# Autodesk Inventor assembly: AS_GENERAL
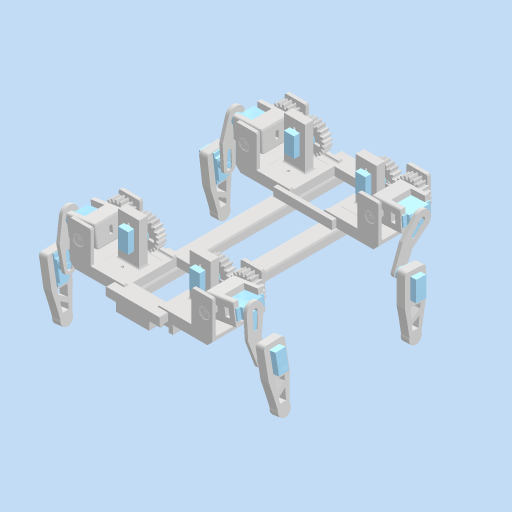
[picture p0: Inventor's stored thumbnail of the model, 512x512]
Saved by Autodesk Inventor 2024 (Build 280153000, 153)
## iProperties
Created: 2024-09-28
Part Number: AS_GENERAL
Document SubType Name: Assembly
Designer: MxMon
Author: MxMon
## Documents named in this file (22)
- C:\Users\MxMon\Documents\Inventor\CHEWIETRON\AS_GENERAL.iam
- C:\Users\MxMon\Documents\Inventor\CHEWIETRON\BASEPRINCIPAL_PATA_IZQ.ipt
- C:\Users\MxMon\Documents\Inventor\CHEWIETRON\bearing_604zz\bearing_604zz.ipt
- C:\Users\MxMon\Documents\Inventor\CHEWIETRON\BASEMOTOR_HOMBRO.ipt
- C:\Users\MxMon\Documents\Inventor\CHEWIETRON\Servo mockup\Servo mockup.ipt
- C:\Users\MxMon\Documents\Inventor\CHEWIETRON\Servo Motor hélice\Servo Motor hélice.ipt
- C:\Users\MxMon\Documents\Inventor\CHEWIETRON\PATA_SUP_IZQ.ipt
- C:\Users\MxMon\Documents\Inventor\CHEWIETRON\PARA_INF.ipt
- C:\Users\MxMon\Documents\Inventor\CHEWIETRON\BASEMOTOR_ENGRANE.ipt
- C:\Users\MxMon\Documents\Inventor\CHEWIETRON\CONECTOR_ENGRANE_HOMBRO.ipt
- C:\Users\MxMon\Documents\Inventor\CHEWIETRON\ENGRANE_HOMBRO.ipt
- C:\Users\MxMon\Documents\Inventor\CHEWIETRON\HELICE_CRUZ.ipt
- C:\Users\MxMon\Documents\Inventor\CHEWIETRON\ENGRANE_HELICE.ipt
- C:\Users\MxMon\Documents\Inventor\CHEWIETRON\EJE_TORNILLO.ipt
- C:\Users\MxMon\Documents\Inventor\CHEWIETRON\TUERCA.ipt
- C:\Users\MxMon\Documents\Inventor\CHEWIETRON\ESPACIADOR.ipt
- C:\Users\MxMon\Documents\Inventor\CHEWIETRON\BASE_DE_PRUEBA.ipt
- C:\Users\MxMon\Documents\Inventor\CHEWIETRON\BASEPRINCIPAL_PATA_DER.ipt
- C:\Users\MxMon\Documents\Inventor\CHEWIETRON\PATA_SUP_DER.ipt
- C:\Users\MxMon\Documents\Inventor\CHEWIETRON\UNION_CHEWIE.ipt
- C:\Users\MxMon\Documents\Inventor\CHEWIETRON\UNION_INTERNA.ipt
- C:\Users\MxMon\Documents\Inventor\CHEWIETRON\TAG.ipt
## Components (83 placed, 21 different names)
1. BASEPRINCIPAL_PATA_IZQ:1 — Mate:1, Mate:2, Mate:3, Mate:4, Mate:23, Mate:25, Mate:46, Mate:98, Mate:129, Mate:149, Flush:2, Mate:150, Mate:201, Mate:202, Mate:210, Mate:211
2. bearing_604zz:1 — Mate:1, Mate:2, Mate:5, Mate:39, Mate:40
3. bearing_604zz:2 — Mate:3, Mate:4, Mate:44
4. BASEMOTOR_HOMBRO:1 — Mate:5, Mate:6, Mate:7, Mate:8, Mate:26, Mate:27, Mate:28, Mate:42
5. Servo mockup:1 — Mate:6, Mate:7, Mate:8, Mate:9, Mate:10
6. Servo Motor hélice:1 — Mate:9, Mate:10, Mate:11, Mate:12, Mate:13
7. PATA_SUP_IZQ:1 — Mate:11, Mate:12, Mate:13, Mate:47, Mate:48, Mate:49, Mate:50
8. Servo mockup:2 — Mate:20, Mate:21, Mate:22
9. Servo Motor hélice:2 — Mate:47, Mate:48, Mate:49, Mate:50
10. PARA_INF:1 — Mate:20, Mate:21, Mate:22
11. BASEMOTOR_ENGRANE:1 — Mate:23, Mate:25, Mate:36, Mate:37, Mate:38, Mate:46
12. CONECTOR_ENGRANE_HOMBRO:1 — Mate:26, Mate:27, Mate:28, Mate:29, Mate:30, Mate:31
13. ENGRANE_HOMBRO:1 — Mate:29, Mate:30, Mate:31
14. Servo mockup:3 — Mate:32, Mate:33, Mate:36, Mate:37, Mate:38
15. HELICE_CRUZ:1 — Mate:32, Mate:33, Mate:34, Mate:35
16. ENGRANE_HELICE:1 — Mate:34, Mate:35
17. EJE_TORNILLO:1 — Mate:39, Mate:40, Mate:41, Mate:43
18. TUERCA:1 — Mate:41, Mate:42, Mate:45
19. ESPACIADOR:1 — Mate:43, Mate:44, Mate:45
20. BASEPRINCIPAL_PATA_IZQ:2 — Mate:97, Mate:99, Flush:1, Mate:130, Mate:131, Mate:205, Mate:206, Mate:212, Mate:213, Mate:214, Mate:216
21. bearing_604zz:3
22. bearing_604zz:4
23. BASEMOTOR_HOMBRO:2
24. Servo mockup:4
25. Servo Motor hélice:3
26. PATA_SUP_IZQ:2
27. Servo mockup:5
28. Servo Motor hélice:4
29. PARA_INF:2
30. BASEMOTOR_ENGRANE:2
31. CONECTOR_ENGRANE_HOMBRO:2
32. ENGRANE_HOMBRO:2
33. Servo mockup:6
34. HELICE_CRUZ:2
35. ENGRANE_HELICE:2
36. EJE_TORNILLO:2
37. TUERCA:2
38. ESPACIADOR:2
39. BASE_DE_PRUEBA:1 — Mate:97, Mate:98, Mate:99, Mate:129
40. BASEPRINCIPAL_PATA_DER:1 — Flush:1, Mate:101, Mate:102, Mate:103, Mate:111, Mate:112, Mate:113, Mate:114, Mate:130, Mate:131, Mate:207, Mate:215
41. BASEMOTOR_ENGRANE:3 — Mate:101, Mate:102, Mate:103, Mate:104, Mate:105, Mate:106
42. Servo mockup:7 — Mate:104, Mate:105, Mate:106, Mate:107, Mate:108
43. HELICE_CRUZ:3 — Mate:107, Mate:108, Mate:109, Mate:110
44. ENGRANE_HELICE:3 — Mate:109, Mate:110
45. bearing_604zz:5 — Mate:111, Mate:112, Mate:116
46. bearing_604zz:6 — Mate:113, Mate:114, Mate:115, Mate:132
47. EJE_TORNILLO:3 — Mate:115, Mate:116, Mate:124, Mate:125, Mate:127
48. BASEMOTOR_HOMBRO:3 — Mate:118, Mate:119, Mate:120, Mate:124, Mate:126, Mate:133, Mate:134, Mate:137
49. CONECTOR_ENGRANE_HOMBRO:3 — Mate:118, Mate:119, Mate:120, Mate:121, Mate:122, Mate:123
50. ENGRANE_HOMBRO:3 — Mate:121, Mate:122, Mate:123
51. TUERCA:3 — Mate:125, Mate:126, Mate:128
52. ESPACIADOR:3 — Mate:127, Mate:128, Mate:132
53. Servo mockup:8 — Mate:133, Mate:134, Mate:135, Mate:136, Mate:137
54. Servo Motor hélice:5 — Mate:135, Mate:136, Mate:138, Mate:139, Mate:140
55. PATA_SUP_DER:1 — Mate:138, Mate:139, Mate:140, Mate:143, Mate:144, Mate:145
56. Servo mockup:9 — Mate:146, Mate:147, Mate:148
57. Servo Motor hélice:6 — Mate:143, Mate:144, Mate:145
58. PARA_INF:3 — Mate:146, Mate:147, Mate:148
59. BASEPRINCIPAL_PATA_DER:2 — Mate:149, Flush:2, Mate:150, Mate:151, Mate:152, Mate:153, Mate:161, Mate:164, Mate:165, Mate:197, Mate:198, Mate:199, Mate:203, Mate:204, Mate:208, Mate:209
60. BASEMOTOR_ENGRANE:4 — Mate:151, Mate:152, Mate:153, Mate:154, Mate:155, Mate:156
61. Servo mockup:10 — Mate:154, Mate:155, Mate:156, Mate:157, Mate:158
62. HELICE_CRUZ:4 — Mate:157, Mate:158, Mate:159, Mate:160
63. ENGRANE_HELICE:4 — Mate:159, Mate:160
64. EJE_TORNILLO:4 — Mate:161, Mate:162, Mate:163, Mate:166, Mate:167, Mate:174, Mate:176
65. bearing_604zz:7 — Mate:163, Mate:165, Mate:166
66. bearing_604zz:8 — Mate:162, Mate:164, Mate:178
67. BASEMOTOR_HOMBRO:4 — Mate:167, Mate:168, Mate:169, Mate:170, Mate:175, Mate:183, Mate:184, Mate:185
68. CONECTOR_ENGRANE_HOMBRO:4 — Mate:168, Mate:169, Mate:170, Mate:171, Mate:172, Mate:173
69. ENGRANE_HOMBRO:4 — Mate:171, Mate:172, Mate:173
70. TUERCA:4 — Mate:174, Mate:175, Mate:177
71. ESPACIADOR:4 — Mate:176, Mate:177, Mate:178
72. Servo mockup:11 — Mate:181, Mate:182, Mate:183, Mate:184, Mate:185
73. PATA_SUP_DER:2 — Mate:186, Mate:187, Mate:188, Mate:191, Mate:192, Mate:193
74. Servo Motor hélice:7 — Mate:181, Mate:182, Mate:186, Mate:187, Mate:188
75. Servo mockup:12 — Mate:194, Mate:195, Mate:196
76. Servo Motor hélice:8 — Mate:191, Mate:192, Mate:193
77. PARA_INF:4 — Mate:194, Mate:195, Mate:196
78. BASE_DE_PRUEBA:2 — Mate:197, Mate:198, Mate:199
79. UNION_CHEWIE:1 — Mate:201, Mate:202, Mate:203, Mate:204, Mate:217, Mate:218, Mate:219
80. UNION_INTERNA:1 — Mate:205, Mate:206, Mate:207, Mate:212
81. UNION_INTERNA:2 — Mate:208, Mate:209, Mate:210, Mate:211
82. UNION_CHEWIE:2 — Mate:213, Mate:214, Mate:215, Mate:216
83. TAG:1 — Mate:217, Mate:218, Mate:219
## Relationships (210: Mate 208, Flush 2)
- Mate:1: BASEPRINCIPAL_PATA_IZQ:1 ↔ bearing_604zz:1
- Mate:2: BASEPRINCIPAL_PATA_IZQ:1 ↔ bearing_604zz:1
- Mate:3: BASEPRINCIPAL_PATA_IZQ:1 ↔ bearing_604zz:2
- Mate:4: BASEPRINCIPAL_PATA_IZQ:1 ↔ bearing_604zz:2
- Mate:5: bearing_604zz:1 ↔ BASEMOTOR_HOMBRO:1
- Mate:6: BASEMOTOR_HOMBRO:1 ↔ Servo mockup:1
- Mate:7: BASEMOTOR_HOMBRO:1 ↔ Servo mockup:1
- Mate:8: BASEMOTOR_HOMBRO:1 ↔ Servo mockup:1
- Mate:9: Servo mockup:1 ↔ Servo Motor hélice:1
- Mate:10: Servo mockup:1 ↔ Servo Motor hélice:1
- Mate:11: Servo Motor hélice:1 ↔ PATA_SUP_IZQ:1
- Mate:12: Servo Motor hélice:1 ↔ PATA_SUP_IZQ:1
- Mate:13: Servo Motor hélice:1 ↔ PATA_SUP_IZQ:1
- [Mate]: Servo mockup:2 ↔ Servo Motor hélice:2
- [Mate]: Servo mockup:2 ↔ Servo Motor hélice:2
- Mate:20: Servo mockup:2 ↔ PARA_INF:1
- Mate:21: Servo mockup:2 ↔ PARA_INF:1
- Mate:22: Servo mockup:2 ↔ PARA_INF:1
- Mate:23: BASEPRINCIPAL_PATA_IZQ:1 ↔ BASEMOTOR_ENGRANE:1
- Mate:25: BASEPRINCIPAL_PATA_IZQ:1 ↔ BASEMOTOR_ENGRANE:1
- Mate:26: BASEMOTOR_HOMBRO:1 ↔ CONECTOR_ENGRANE_HOMBRO:1
- Mate:27: BASEMOTOR_HOMBRO:1 ↔ CONECTOR_ENGRANE_HOMBRO:1
- Mate:28: BASEMOTOR_HOMBRO:1 ↔ CONECTOR_ENGRANE_HOMBRO:1
- Mate:29: CONECTOR_ENGRANE_HOMBRO:1 ↔ ENGRANE_HOMBRO:1
- Mate:30: CONECTOR_ENGRANE_HOMBRO:1 ↔ ENGRANE_HOMBRO:1
- Mate:31: CONECTOR_ENGRANE_HOMBRO:1 ↔ ENGRANE_HOMBRO:1
- Mate:32: Servo mockup:3 ↔ HELICE_CRUZ:1
- Mate:33: Servo mockup:3 ↔ HELICE_CRUZ:1
- Mate:34: HELICE_CRUZ:1 ↔ ENGRANE_HELICE:1
- Mate:35: HELICE_CRUZ:1 ↔ ENGRANE_HELICE:1
- Mate:36: BASEMOTOR_ENGRANE:1 ↔ Servo mockup:3
- Mate:37: BASEMOTOR_ENGRANE:1 ↔ Servo mockup:3
- Mate:38: BASEMOTOR_ENGRANE:1 ↔ Servo mockup:3
- Mate:39: bearing_604zz:1 ↔ EJE_TORNILLO:1
- Mate:40: bearing_604zz:1 ↔ EJE_TORNILLO:1
- Mate:41: EJE_TORNILLO:1 ↔ TUERCA:1
- Mate:42: BASEMOTOR_HOMBRO:1 ↔ TUERCA:1
- Mate:43: EJE_TORNILLO:1 ↔ ESPACIADOR:1
- Mate:44: bearing_604zz:2 ↔ ESPACIADOR:1
- Mate:45: TUERCA:1 ↔ ESPACIADOR:1
- Mate:46: BASEPRINCIPAL_PATA_IZQ:1 ↔ BASEMOTOR_ENGRANE:1
- Mate:47: PATA_SUP_IZQ:1 ↔ Servo Motor hélice:2
- Mate:48: PATA_SUP_IZQ:1 ↔ Servo Motor hélice:2
- Mate:49: PATA_SUP_IZQ:1 ↔ Servo Motor hélice:2
- Mate:50: PATA_SUP_IZQ:1 ↔ Servo Motor hélice:2
- [Mate]: BASEPRINCIPAL_PATA_IZQ:2 ↔ bearing_604zz:3
- [Mate]: BASEPRINCIPAL_PATA_IZQ:2 ↔ bearing_604zz:3
- [Mate]: BASEPRINCIPAL_PATA_IZQ:2 ↔ bearing_604zz:4
- [Mate]: BASEPRINCIPAL_PATA_IZQ:2 ↔ bearing_604zz:4
- [Mate]: bearing_604zz:3 ↔ BASEMOTOR_HOMBRO:2
- [Mate]: BASEMOTOR_HOMBRO:2 ↔ Servo mockup:4
- [Mate]: BASEMOTOR_HOMBRO:2 ↔ Servo mockup:4
- [Mate]: BASEMOTOR_HOMBRO:2 ↔ Servo mockup:4
- [Mate]: Servo mockup:4 ↔ Servo Motor hélice:3
- [Mate]: Servo mockup:4 ↔ Servo Motor hélice:3
- [Mate]: Servo Motor hélice:3 ↔ PATA_SUP_IZQ:2
- [Mate]: Servo Motor hélice:3 ↔ PATA_SUP_IZQ:2
- [Mate]: Servo Motor hélice:3 ↔ PATA_SUP_IZQ:2
- [Mate]: Servo mockup:5 ↔ Servo Motor hélice:4
- [Mate]: Servo mockup:5 ↔ Servo Motor hélice:4
- [Mate]: Servo mockup:5 ↔ PARA_INF:2
- [Mate]: Servo mockup:5 ↔ PARA_INF:2
- [Mate]: Servo mockup:5 ↔ PARA_INF:2
- [Mate]: BASEPRINCIPAL_PATA_IZQ:2 ↔ BASEMOTOR_ENGRANE:2
- [Mate]: BASEPRINCIPAL_PATA_IZQ:2 ↔ BASEMOTOR_ENGRANE:2
- [Mate]: BASEMOTOR_HOMBRO:2 ↔ CONECTOR_ENGRANE_HOMBRO:2
- [Mate]: BASEMOTOR_HOMBRO:2 ↔ CONECTOR_ENGRANE_HOMBRO:2
- [Mate]: BASEMOTOR_HOMBRO:2 ↔ CONECTOR_ENGRANE_HOMBRO:2
- [Mate]: CONECTOR_ENGRANE_HOMBRO:2 ↔ ENGRANE_HOMBRO:2
- [Mate]: CONECTOR_ENGRANE_HOMBRO:2 ↔ ENGRANE_HOMBRO:2
- [Mate]: CONECTOR_ENGRANE_HOMBRO:2 ↔ ENGRANE_HOMBRO:2
- [Mate]: Servo mockup:6 ↔ HELICE_CRUZ:2
- [Mate]: Servo mockup:6 ↔ HELICE_CRUZ:2
- [Mate]: HELICE_CRUZ:2 ↔ ENGRANE_HELICE:2
- [Mate]: HELICE_CRUZ:2 ↔ ENGRANE_HELICE:2
- [Mate]: BASEMOTOR_ENGRANE:2 ↔ Servo mockup:6
- [Mate]: BASEMOTOR_ENGRANE:2 ↔ Servo mockup:6
- [Mate]: BASEMOTOR_ENGRANE:2 ↔ Servo mockup:6
- [Mate]: bearing_604zz:3 ↔ EJE_TORNILLO:2
- [Mate]: bearing_604zz:3 ↔ EJE_TORNILLO:2
- [Mate]: EJE_TORNILLO:2 ↔ TUERCA:2
- [Mate]: BASEMOTOR_HOMBRO:2 ↔ TUERCA:2
- [Mate]: EJE_TORNILLO:2 ↔ ESPACIADOR:2
- [Mate]: bearing_604zz:4 ↔ ESPACIADOR:2
- [Mate]: TUERCA:2 ↔ ESPACIADOR:2
- [Mate]: BASEPRINCIPAL_PATA_IZQ:2 ↔ BASEMOTOR_ENGRANE:2
- [Mate]: PATA_SUP_IZQ:2 ↔ Servo Motor hélice:4
- [Mate]: PATA_SUP_IZQ:2 ↔ Servo Motor hélice:4
- [Mate]: PATA_SUP_IZQ:2 ↔ Servo Motor hélice:4
- [Mate]: PATA_SUP_IZQ:2 ↔ Servo Motor hélice:4
- Mate:97: BASEPRINCIPAL_PATA_IZQ:2 ↔ BASE_DE_PRUEBA:1
- Mate:98: BASEPRINCIPAL_PATA_IZQ:1 ↔ BASE_DE_PRUEBA:1
- Mate:99: BASEPRINCIPAL_PATA_IZQ:2 ↔ BASE_DE_PRUEBA:1
- Flush:1: BASEPRINCIPAL_PATA_IZQ:2 ↔ BASEPRINCIPAL_PATA_DER:1
- Mate:101: BASEPRINCIPAL_PATA_DER:1 ↔ BASEMOTOR_ENGRANE:3
- Mate:102: BASEPRINCIPAL_PATA_DER:1 ↔ BASEMOTOR_ENGRANE:3
- Mate:103: BASEPRINCIPAL_PATA_DER:1 ↔ BASEMOTOR_ENGRANE:3
- Mate:104: BASEMOTOR_ENGRANE:3 ↔ Servo mockup:7
- Mate:105: BASEMOTOR_ENGRANE:3 ↔ Servo mockup:7
- Mate:106: BASEMOTOR_ENGRANE:3 ↔ Servo mockup:7
- Mate:107: Servo mockup:7 ↔ HELICE_CRUZ:3
- Mate:108: Servo mockup:7 ↔ HELICE_CRUZ:3
- Mate:109: HELICE_CRUZ:3 ↔ ENGRANE_HELICE:3
- Mate:110: HELICE_CRUZ:3 ↔ ENGRANE_HELICE:3
- Mate:111: BASEPRINCIPAL_PATA_DER:1 ↔ bearing_604zz:5
- Mate:112: BASEPRINCIPAL_PATA_DER:1 ↔ bearing_604zz:5
- Mate:113: BASEPRINCIPAL_PATA_DER:1 ↔ bearing_604zz:6
- Mate:114: BASEPRINCIPAL_PATA_DER:1 ↔ bearing_604zz:6
- Mate:115: bearing_604zz:6 ↔ EJE_TORNILLO:3
- Mate:116: bearing_604zz:5 ↔ EJE_TORNILLO:3
- Mate:118: BASEMOTOR_HOMBRO:3 ↔ CONECTOR_ENGRANE_HOMBRO:3
- Mate:119: BASEMOTOR_HOMBRO:3 ↔ CONECTOR_ENGRANE_HOMBRO:3
- Mate:120: BASEMOTOR_HOMBRO:3 ↔ CONECTOR_ENGRANE_HOMBRO:3
- Mate:121: CONECTOR_ENGRANE_HOMBRO:3 ↔ ENGRANE_HOMBRO:3
- Mate:122: CONECTOR_ENGRANE_HOMBRO:3 ↔ ENGRANE_HOMBRO:3
- Mate:123: CONECTOR_ENGRANE_HOMBRO:3 ↔ ENGRANE_HOMBRO:3
- Mate:124: EJE_TORNILLO:3 ↔ BASEMOTOR_HOMBRO:3
- Mate:125: EJE_TORNILLO:3 ↔ TUERCA:3
- Mate:126: BASEMOTOR_HOMBRO:3 ↔ TUERCA:3
- Mate:127: EJE_TORNILLO:3 ↔ ESPACIADOR:3
- Mate:128: TUERCA:3 ↔ ESPACIADOR:3
- Mate:129: BASEPRINCIPAL_PATA_IZQ:1 ↔ BASE_DE_PRUEBA:1
- Mate:130 (40 mm): BASEPRINCIPAL_PATA_IZQ:2 ↔ BASEPRINCIPAL_PATA_DER:1
- Mate:131: BASEPRINCIPAL_PATA_IZQ:2 ↔ BASEPRINCIPAL_PATA_DER:1
- Mate:132: bearing_604zz:6 ↔ ESPACIADOR:3
- Mate:133: BASEMOTOR_HOMBRO:3 ↔ Servo mockup:8
- Mate:134: BASEMOTOR_HOMBRO:3 ↔ Servo mockup:8
- Mate:135: Servo mockup:8 ↔ Servo Motor hélice:5
- Mate:136: Servo mockup:8 ↔ Servo Motor hélice:5
- Mate:137: BASEMOTOR_HOMBRO:3 ↔ Servo mockup:8
- Mate:138: Servo Motor hélice:5 ↔ PATA_SUP_DER:1
- Mate:139: Servo Motor hélice:5 ↔ PATA_SUP_DER:1
- Mate:140: Servo Motor hélice:5 ↔ PATA_SUP_DER:1
- [Mate]: Servo mockup:9 ↔ Servo Motor hélice:6
- [Mate]: Servo mockup:9 ↔ Servo Motor hélice:6
- Mate:143: PATA_SUP_DER:1 ↔ Servo Motor hélice:6
- Mate:144: PATA_SUP_DER:1 ↔ Servo Motor hélice:6
- Mate:145: PATA_SUP_DER:1 ↔ Servo Motor hélice:6
- Mate:146: Servo mockup:9 ↔ PARA_INF:3
- Mate:147: Servo mockup:9 ↔ PARA_INF:3
- Mate:148: Servo mockup:9 ↔ PARA_INF:3
- Mate:149 (40 mm): BASEPRINCIPAL_PATA_IZQ:1 ↔ BASEPRINCIPAL_PATA_DER:2
- Flush:2: BASEPRINCIPAL_PATA_IZQ:1 ↔ BASEPRINCIPAL_PATA_DER:2
- Mate:150: BASEPRINCIPAL_PATA_IZQ:1 ↔ BASEPRINCIPAL_PATA_DER:2
- Mate:151: BASEPRINCIPAL_PATA_DER:2 ↔ BASEMOTOR_ENGRANE:4
- Mate:152: BASEPRINCIPAL_PATA_DER:2 ↔ BASEMOTOR_ENGRANE:4
- Mate:153: BASEPRINCIPAL_PATA_DER:2 ↔ BASEMOTOR_ENGRANE:4
- Mate:154: BASEMOTOR_ENGRANE:4 ↔ Servo mockup:10
- Mate:155: BASEMOTOR_ENGRANE:4 ↔ Servo mockup:10
- Mate:156: BASEMOTOR_ENGRANE:4 ↔ Servo mockup:10
- Mate:157: Servo mockup:10 ↔ HELICE_CRUZ:4
- Mate:158: Servo mockup:10 ↔ HELICE_CRUZ:4
- Mate:159: HELICE_CRUZ:4 ↔ ENGRANE_HELICE:4
- Mate:160: HELICE_CRUZ:4 ↔ ENGRANE_HELICE:4
- Mate:161: BASEPRINCIPAL_PATA_DER:2 ↔ EJE_TORNILLO:4
- Mate:162: EJE_TORNILLO:4 ↔ bearing_604zz:8
- Mate:163: EJE_TORNILLO:4 ↔ bearing_604zz:7
- Mate:164: BASEPRINCIPAL_PATA_DER:2 ↔ bearing_604zz:8
- Mate:165: BASEPRINCIPAL_PATA_DER:2 ↔ bearing_604zz:7
- Mate:166: EJE_TORNILLO:4 ↔ bearing_604zz:7
- Mate:167: EJE_TORNILLO:4 ↔ BASEMOTOR_HOMBRO:4
- Mate:168: BASEMOTOR_HOMBRO:4 ↔ CONECTOR_ENGRANE_HOMBRO:4
- Mate:169: BASEMOTOR_HOMBRO:4 ↔ CONECTOR_ENGRANE_HOMBRO:4
- Mate:170: BASEMOTOR_HOMBRO:4 ↔ CONECTOR_ENGRANE_HOMBRO:4
- Mate:171: CONECTOR_ENGRANE_HOMBRO:4 ↔ ENGRANE_HOMBRO:4
- Mate:172: CONECTOR_ENGRANE_HOMBRO:4 ↔ ENGRANE_HOMBRO:4
- Mate:173: CONECTOR_ENGRANE_HOMBRO:4 ↔ ENGRANE_HOMBRO:4
- Mate:174: EJE_TORNILLO:4 ↔ TUERCA:4
- Mate:175: BASEMOTOR_HOMBRO:4 ↔ TUERCA:4
- Mate:176: EJE_TORNILLO:4 ↔ ESPACIADOR:4
- Mate:177: TUERCA:4 ↔ ESPACIADOR:4
- Mate:178: bearing_604zz:8 ↔ ESPACIADOR:4
- Mate:181: Servo mockup:11 ↔ Servo Motor hélice:7
- Mate:182: Servo mockup:11 ↔ Servo Motor hélice:7
- Mate:183: BASEMOTOR_HOMBRO:4 ↔ Servo mockup:11
- Mate:184: BASEMOTOR_HOMBRO:4 ↔ Servo mockup:11
- Mate:185: BASEMOTOR_HOMBRO:4 ↔ Servo mockup:11
- Mate:186: PATA_SUP_DER:2 ↔ Servo Motor hélice:7
- Mate:187: PATA_SUP_DER:2 ↔ Servo Motor hélice:7
- Mate:188: PATA_SUP_DER:2 ↔ Servo Motor hélice:7
- [Mate]: Servo mockup:12 ↔ Servo Motor hélice:8
- [Mate]: Servo mockup:12 ↔ Servo Motor hélice:8
- Mate:191: PATA_SUP_DER:2 ↔ Servo Motor hélice:8
- Mate:192: PATA_SUP_DER:2 ↔ Servo Motor hélice:8
- Mate:193: PATA_SUP_DER:2 ↔ Servo Motor hélice:8
- Mate:194: Servo mockup:12 ↔ PARA_INF:4
- Mate:195: Servo mockup:12 ↔ PARA_INF:4
- Mate:196: Servo mockup:12 ↔ PARA_INF:4
- Mate:197: BASEPRINCIPAL_PATA_DER:2 ↔ BASE_DE_PRUEBA:2
- Mate:198: BASEPRINCIPAL_PATA_DER:2 ↔ BASE_DE_PRUEBA:2
- Mate:199: BASEPRINCIPAL_PATA_DER:2 ↔ BASE_DE_PRUEBA:2
- Mate:201: BASEPRINCIPAL_PATA_IZQ:1 ↔ UNION_CHEWIE:1
- Mate:202: BASEPRINCIPAL_PATA_IZQ:1 ↔ UNION_CHEWIE:1
- Mate:203: BASEPRINCIPAL_PATA_DER:2 ↔ UNION_CHEWIE:1
- Mate:204: BASEPRINCIPAL_PATA_DER:2 ↔ UNION_CHEWIE:1
- Mate:205: BASEPRINCIPAL_PATA_IZQ:2 ↔ UNION_INTERNA:1
- Mate:206: BASEPRINCIPAL_PATA_IZQ:2 ↔ UNION_INTERNA:1
- Mate:207: BASEPRINCIPAL_PATA_DER:1 ↔ UNION_INTERNA:1
- Mate:208: BASEPRINCIPAL_PATA_DER:2 ↔ UNION_INTERNA:2
- Mate:209: BASEPRINCIPAL_PATA_DER:2 ↔ UNION_INTERNA:2
- Mate:210: BASEPRINCIPAL_PATA_IZQ:1 ↔ UNION_INTERNA:2
- Mate:211: BASEPRINCIPAL_PATA_IZQ:1 ↔ UNION_INTERNA:2
- Mate:212: BASEPRINCIPAL_PATA_IZQ:2 ↔ UNION_INTERNA:1
- Mate:213: BASEPRINCIPAL_PATA_IZQ:2 ↔ UNION_CHEWIE:2
- Mate:214: BASEPRINCIPAL_PATA_IZQ:2 ↔ UNION_CHEWIE:2
- Mate:215: BASEPRINCIPAL_PATA_DER:1 ↔ UNION_CHEWIE:2
- Mate:216: BASEPRINCIPAL_PATA_IZQ:2 ↔ UNION_CHEWIE:2
- Mate:217: UNION_CHEWIE:1 ↔ TAG:1
- Mate:218 (5 mm): UNION_CHEWIE:1 ↔ TAG:1
- Mate:219 (2.5 mm): UNION_CHEWIE:1 ↔ TAG:1
## Named parameters: d16_d8 = 0 mm, d17_d9 = 0 mm, d57_d0 = 0 mm, d58_d1 = 0 mm, d59_d2 = 0 mm, d60_d3 = 0 mm, d61_d4 = 0 mm, d62_d5 = 0 mm, d63_d6 = 0 mm, d64_d7 = 0 mm, d65_d8 = 0 mm, d66_d9 = 0 mm, d67_d12 = 0 mm, d68_d24 = 0 mm, d69_d25 = 0 mm, d70_d26 = 0 mm, d71_d27 = 0 mm, d72_d29 = 0 mm, d73_d30 = 0 mm, d74_d31 = 0 mm, d75_d32 = 0 mm, d76_d33 = 0 mm, d77_d34 = 0 mm, d78_d35 = 0 mm, d79_d14 = 0 mm, d80_d15 = 0 mm, d81_d16_d8 = 0 mm, d82_d17_d9 = 0 mm, d83_d36 = 0 mm, d84_d37 = 0 mm, d85_d38 = 0 mm, d86_d39 = 0 mm, d87_d40 = 0 mm, d88_d41 = 0 mm, d89_d42 = 0 mm, d90_d43 = 0 mm, d91_d44 = 0 mm, d92_d45 = 0 mm, d93_d46 = 0 mm, d94_d47 = 0 mm, d95_d48 = 0 mm, d96_d49 = 0 mm, d97_d50 = 0 mm, d98_d51 = 0 mm, d99_d53 = 0 mm, d100_d54 = 0 mm, d101_d55 = 0 mm, d209_d203 = 0 mm, d210_d204 = 0 mm, d264_d255 = 0 mm, d265_d256 = 0 mm
